# Autodesk Inventor assembly: fc16-114
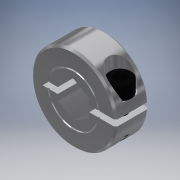
[picture p0: Inventor's stored thumbnail of the model, 180x180]
Saved by Autodesk Inventor 2017.1 (Build 211199000, 199)
## iProperties
Category: Miscellaneous
Company: Autodesk Inc.
Created: 2016-12-20
Part Number: fc16-114
Document SubType Name: Assembly
Designer: Autodesk Inc.
Catalog Web Link: http://www.ruland.com/shaft-collar.php?recordID=CL-6HX-A
Vendor: Ruland
Author: Autodesk Inc.
Keywords: FIRST Choice
## Documents named in this file (3)
- D:\FIRST\FIRST KOP 2017\FIRST FirstChoice 2017\fc17-114_ShaftCollar.iam
- D:\FIRST\FIRST KOP 2017\FIRST FirstChoice 2017\Parts\MISC_ShaftCollar_CL-6HX-A.ipt
- D:\FIRST\FIRST KOP 2017\FIRST FirstChoice 2017\Parts\ANSI B18.3 - 6-32 UNC - 0.375(31).ipt
## Components (2 placed, 2 different names)
1. MISC_ShaftCollar_CL-6HX-A:1 — Insert:1
2. Hexagon Socket Head Cap Screw - Inch No. 6 - 32 UNC - 3/8:1 — Insert:1
## Relationships (1: Insert 1)
- Insert:1: MISC_ShaftCollar_CL-6HX-A:1 ↔ Hexagon Socket Head Cap Screw - Inch No. 6 - 32 UNC - 3/8:1
